# Autodesk Inventor assembly: FastBattery2
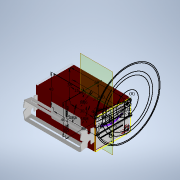
[picture p0: Inventor's stored thumbnail of the model, 180x180]
Saved by Autodesk Inventor 2022 (Build 260153000, 153)
## iProperties
Created: 2024-07-22
Part Number: FastBattery2
Document SubType Name: Assembly
Designer: Капустяник Андрей
Author: Капустяник Андрей
## Documents named in this file (15)
- C:\Users\akap\Documents\Git\MZCAT_2024_construction\MZCAT_battery\FastBattery2.iam
- C:\Users\akap\Documents\Git\MZCAT_2024_construction\MZCAT_battery\plan.ipt
- C:\Users\akap\Documents\Git\MZCAT_2024_construction\MZCAT_battery\Bat18650.ipt
- C:\Users\akap\Documents\Git\MZCAT_2024_construction\MZCAT_battery\battery_header 7P.ipt
- C:\Users\akap\Documents\Git\MZCAT_2024_construction\MZCAT_battery\xb-acf005-2r.ipt
- C:\Users\akap\Documents\Git\MZCAT_2024_construction\MZCAT_battery\BMS_board.ipt
- C:\Users\akap\Documents\Git\MZCAT_2024_construction\MZCAT_battery\ButerBoard.ipt
- C:\Users\akap\Documents\Git\MZCAT_2024_construction\MZCAT_battery\User Library-User Library-DFN5x6_SO8FL-1.ipt
- C:\Users\akap\Documents\Git\MZCAT_2024_construction\MZCAT_battery\investment nut M2 OD3,2 L2,5.ipt
- C:\Users\akap\Documents\Git\MZCAT_2024_construction\MZCAT_battery\M2 4mm HEX.ipt
- C:\Users\akap\Documents\Git\MZCAT_2024_construction\MZCAT_battery\akkum_base2_1.ipt
- C:\Users\akap\Documents\Git\MZCAT_2024_construction\MZCAT_battery\akkum_base2_2.ipt
- C:\Users\akap\Documents\Git\MZCAT_2024_construction\MZCAT_battery\petal_fixed.ipt
- C:\Users\akap\Documents\Git\MZCAT_2024_construction\MZCAT_battery\metal_body_fixed.ipt
- C:\Users\akap\Documents\Git\MZCAT_2024_construction\MZCAT_battery\metal_cap_fixed.ipt
## Components (28 placed, 14 different names)
1. plan:1 — Заподлицо:1, Заподлицо:2, Заподлицо:3, Совмещение:4, Совмещение:5, Совмещение:6, Совмещение:9
2. Bat18650:1 — Заподлицо:4, Совмещение:1, Совмещение:2, Совмещение:6, Совмещение:23, Совмещение:26
3. Bat18650:2 — Заподлицо:5, Совмещение:3, Совмещение:5, Совмещение:24
4. Bat18650:3 — Заподлицо:4, Заподлицо:5, Совмещение:3, Совмещение:4, Совмещение:25
5. battery_header 7P:1 — Совмещение:7, Совмещение:9, Совмещение:12, Совмещение:15
6. xb-acf005-2r:1 — Совмещение:17, Совмещение:18, Совмещение:39
7. BMS_board:1 — Совмещение:7, Совмещение:10, Совмещение:11, Совмещение:12, Совмещение:15, Заподлицо:14, Совмещение:21, Совмещение:22, С поворотом:7, С поворотом:8, С поворотом:9, С поворотом:10
8. ButerBoard:1 — Заподлицо:14, Совмещение:16, Совмещение:17, Совмещение:18, Совмещение:19
9. User Library-User Library-DFN5x6_SO8FL-1:1 — Совмещение:22
10. User Library-User Library-DFN5x6_SO8FL-1:2 — Совмещение:21
11. investment nut M2 OD3,2 L2,5:1 — Заподлицо:23, Совмещение:32, Совмещение:33
12. investment nut M2 OD3,2 L2,5:2 — Заподлицо:24, Совмещение:31, Совмещение:34
13. investment nut M2 OD3,2 L2,5:3 — Совмещение:28, Заподлицо:20
14. investment nut M2 OD3,2 L2,5:4 — Совмещение:29, Заподлицо:22
15. investment nut M2 OD3,2 L2,5:5 — Совмещение:27, Заподлицо:19, Совмещение:35
16. investment nut M2 OD3,2 L2,5:6 — Совмещение:30, Заподлицо:21, Совмещение:36
17. M2 4mm HEX:1 — С поворотом:7, Совмещение:36
18. M2 4mm HEX:2 — Совмещение:34, Совмещение:40
19. M2 4mm HEX:3 — С поворотом:9
20. M2 4mm HEX:4 — Совмещение:33
21. M2 4mm HEX:5 — С поворотом:8
22. M2 4mm HEX:6 — С поворотом:10, Совмещение:35
23. akkum_base2_1:1 — Совмещение:23, Совмещение:24, Совмещение:29, Совмещение:30, Заподлицо:21, Заподлицо:22, Заподлицо:23, Совмещение:32, Совмещение:38
24. akkum_base2_2:1 — Совмещение:25, Совмещение:26, Совмещение:27, Совмещение:28, Заподлицо:19, Заподлицо:20, Заподлицо:24, Совмещение:31, Совмещение:37, Совмещение:42, Совмещение:43
25. petal_fixed:1 — Совмещение:43, Заподлицо:26, Заподлицо:27
26. petal_fixed:2 — Совмещение:42, Заподлицо:26, Заподлицо:27
27. metal_body_fixed:1 — Совмещение:37, Совмещение:38, Совмещение:39, Совмещение:41, Заподлицо:25
28. metal_cap_fixed:1 — Совмещение:40, Совмещение:41, Заподлицо:25
## Relationships (58: Mate 39, Flush 15, RevoluteJoint 4)
- Заподлицо:1 [Flush]: plan:1
- Заподлицо:2 [Flush]: plan:1
- Заподлицо:3 [Flush]: plan:1
- Заподлицо:4 [Flush]: Bat18650:1 ↔ Bat18650:3
- Заподлицо:5 [Flush]: Bat18650:2 ↔ Bat18650:3
- Совмещение:1 [Mate]: Bat18650:1
- Совмещение:2 [Mate]: Bat18650:1
- Совмещение:3 [Mate]: Bat18650:2 ↔ Bat18650:3
- Совмещение:4 [Mate]: plan:1 ↔ Bat18650:3
- Совмещение:5 [Mate]: plan:1 ↔ Bat18650:2
- Совмещение:6 [Mate]: plan:1 ↔ Bat18650:1
- Совмещение:7 [Mate]: battery_header 7P:1 ↔ BMS_board:1
- Совмещение:9 [Mate]: plan:1 ↔ battery_header 7P:1
- Совмещение:10 [Mate]: BMS_board:1
- Совмещение:11 [Mate]: BMS_board:1
- Совмещение:12 [Mate]: battery_header 7P:1 ↔ BMS_board:1
- Совмещение:15 [Mate]: battery_header 7P:1 ↔ BMS_board:1
- Заподлицо:14 [Flush]: BMS_board:1 ↔ ButerBoard:1
- Совмещение:16 [Mate]: ButerBoard:1
- Совмещение:17 [Mate]: xb-acf005-2r:1 ↔ ButerBoard:1
- Совмещение:18 [Mate]: xb-acf005-2r:1 ↔ ButerBoard:1
- Совмещение:19 [Mate] (-10 mm): ButerBoard:1
- Совмещение:21 [Mate]: BMS_board:1 ↔ User Library-User Library-DFN5x6_SO8FL-1:2
- Совмещение:22 [Mate]: BMS_board:1 ↔ User Library-User Library-DFN5x6_SO8FL-1:1
- С поворотом:7 [RevoluteJoint]: BMS_board:1 ↔ M2 4mm HEX:1
- С поворотом:8 [RevoluteJoint]: BMS_board:1 ↔ M2 4mm HEX:5
- С поворотом:9 [RevoluteJoint]: BMS_board:1 ↔ M2 4mm HEX:3
- С поворотом:10 [RevoluteJoint]: BMS_board:1 ↔ M2 4mm HEX:6
- Совмещение:23 [Mate]: Bat18650:1 ↔ akkum_base2_1:1
- Совмещение:24 [Mate]: Bat18650:2 ↔ akkum_base2_1:1
- Совмещение:25 [Mate]: Bat18650:3 ↔ akkum_base2_2:1
- Совмещение:26 [Mate]: Bat18650:1 ↔ akkum_base2_2:1
- Совмещение:27 [Mate]: investment nut M2 OD3,2 L2,5:5 ↔ akkum_base2_2:1
- Совмещение:28 [Mate]: investment nut M2 OD3,2 L2,5:3 ↔ akkum_base2_2:1
- Заподлицо:19 [Flush]: investment nut M2 OD3,2 L2,5:5 ↔ akkum_base2_2:1
- Заподлицо:20 [Flush]: investment nut M2 OD3,2 L2,5:3 ↔ akkum_base2_2:1
- Совмещение:29 [Mate]: investment nut M2 OD3,2 L2,5:4 ↔ akkum_base2_1:1
- Совмещение:30 [Mate]: investment nut M2 OD3,2 L2,5:6 ↔ akkum_base2_1:1
- Заподлицо:21 [Flush]: investment nut M2 OD3,2 L2,5:6 ↔ akkum_base2_1:1
- Заподлицо:22 [Flush]: investment nut M2 OD3,2 L2,5:4 ↔ akkum_base2_1:1
- Заподлицо:23 [Flush]: investment nut M2 OD3,2 L2,5:1 ↔ akkum_base2_1:1
- Заподлицо:24 [Flush]: investment nut M2 OD3,2 L2,5:2 ↔ akkum_base2_2:1
- Совмещение:31 [Mate]: investment nut M2 OD3,2 L2,5:2 ↔ akkum_base2_2:1
- Совмещение:32 [Mate]: investment nut M2 OD3,2 L2,5:1 ↔ akkum_base2_1:1
- Совмещение:33 [Mate]: investment nut M2 OD3,2 L2,5:1 ↔ M2 4mm HEX:4
- Совмещение:34 [Mate]: investment nut M2 OD3,2 L2,5:2 ↔ M2 4mm HEX:2
- Совмещение:35 [Mate]: investment nut M2 OD3,2 L2,5:5 ↔ M2 4mm HEX:6
- Совмещение:36 [Mate]: investment nut M2 OD3,2 L2,5:6 ↔ M2 4mm HEX:1
- Совмещение:37 [Mate]: akkum_base2_2:1 ↔ metal_body_fixed:1
- Совмещение:38 [Mate]: akkum_base2_1:1 ↔ metal_body_fixed:1
- Совмещение:39 [Mate]: xb-acf005-2r:1 ↔ metal_body_fixed:1
- Совмещение:40 [Mate]: M2 4mm HEX:2 ↔ metal_cap_fixed:1
- Совмещение:41 [Mate]: metal_body_fixed:1 ↔ metal_cap_fixed:1
- Заподлицо:25 [Flush]: metal_body_fixed:1 ↔ metal_cap_fixed:1
- Совмещение:42 [Mate]: akkum_base2_2:1 ↔ petal_fixed:2
- Совмещение:43 [Mate]: akkum_base2_2:1 ↔ petal_fixed:1
- Заподлицо:26 [Flush]: petal_fixed:1 ↔ petal_fixed:2
- Заподлицо:27 [Flush]: petal_fixed:1 ↔ petal_fixed:2
